# Autodesk Inventor assembly: Truss4
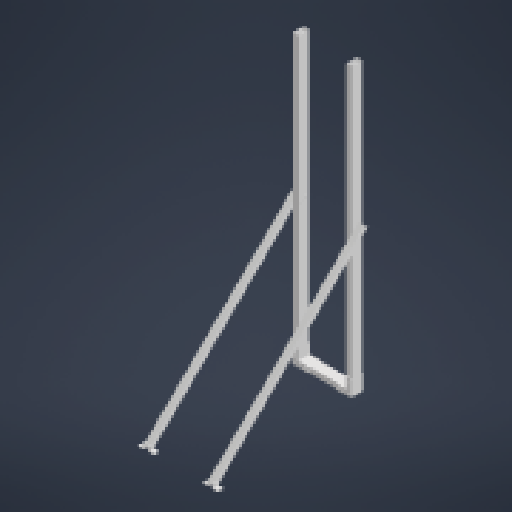
[picture p0: Inventor's stored thumbnail of the model, 512x512]
Saved by Autodesk Inventor 2023 (Build 270158000, 158)
## iProperties
Created: 2023-01-18
Part Number: Truss4
Document SubType Name: Assembly
Designer: Terrence
Author: Terrence
## Documents named in this file (7)
- C:\Users\Terrence\Documents\FRC Long\Truss\Truss4.iam
- C:\Users\Terrence\Documents\FRC Long\Truss\Solid1_2.ipt
- C:\Users\Terrence\Documents\FRC Long\Truss\Solid6_1.ipt
- C:\Users\Terrence\Documents\FRC Long\Truss\Solid7_1.ipt
- C:\Users\Terrence\Documents\FRC Long\Truss\Solid9_1.ipt
- C:\Users\Terrence\Documents\FRC Long\Truss\Solid10_1.ipt
- C:\Users\Terrence\Documents\FRC Long\Truss\Solid11.ipt
## Components (13 placed, 6 different names)
1. Solid1_2:1 — Insert:4, Insert:5
2. Solid6_1:1
3. Solid7_1:1
4. Solid9_1:1
5. Solid10_1:1 — Insert:3, Insert:8, Insert:9
6. Solid11:1
7. Solid1_2:2 — Insert:1, Insert:2, Insert:6, Insert:7, Insert:14, Insert:15
8. Solid9_1:2 — Insert:1, Insert:2, Insert:3, Insert:9
9. Solid9_1:3 — Insert:4, Insert:5
10. Solid9_1:4 — Insert:6, Insert:7, Insert:8
11. Solid6_1:2 — Insert:10, Insert:11, Insert:12, Insert:13, Insert:14, Insert:15
12. Solid7_1:2 — Insert:10, Insert:11
13. Solid11:2 — Insert:12, Insert:13
## Relationships (15: Insert 15)
- Insert:1: Solid1_2:2 ↔ Solid9_1:2
- Insert:2: Solid1_2:2 ↔ Solid9_1:2
- Insert:3: Solid10_1:1 ↔ Solid9_1:2
- Insert:4: Solid1_2:1 ↔ Solid9_1:3
- Insert:5: Solid1_2:1 ↔ Solid9_1:3
- Insert:6: Solid1_2:2 ↔ Solid9_1:4
- Insert:7: Solid1_2:2 ↔ Solid9_1:4
- Insert:8: Solid10_1:1 ↔ Solid9_1:4
- Insert:9: Solid10_1:1 ↔ Solid9_1:2
- Insert:10: Solid6_1:2 ↔ Solid7_1:2
- Insert:11: Solid6_1:2 ↔ Solid7_1:2
- Insert:12: Solid6_1:2 ↔ Solid11:2
- Insert:13: Solid6_1:2 ↔ Solid11:2
- Insert:14: Solid1_2:2 ↔ Solid6_1:2
- Insert:15: Solid1_2:2 ↔ Solid6_1:2
